# Autodesk Inventor assembly: Ensamblaje SCARA
(part 2 of 2)
- Coincidencia:936 [Mate]: ISO 4017 M4 x 40:3 ↔ ISO 4032 M4:2
- Coincidencia:944 [Mate]: Segundo segmento - inferior - Shape generator prueba 2 - 40%:1 ↔ ISO 7045 H M4 x 16 - 4.8 - H:4
- Coincidencia:945 [Mate]: Segundo segmento - inferior - Shape generator prueba 2 - 40%:1 ↔ ISO 7045 H M4 x 16 - 4.8 - H:5
- Coincidencia:946 [Mate]: Segundo segmento - inferior - Shape generator prueba 2 - 40%:1 ↔ ISO 7045 H M4 x 16 - 4.8 - H:3
- Coincidencia:947 [Mate]: Segundo segmento - inferior - Shape generator prueba 2 - 40%:1 ↔ ISO 7045 H M4 x 16 - 4.8 - H:1
- Coincidencia:948 [Mate]: Segundo segmento - inferior - Shape generator prueba 2 - 40%:1 ↔ ISO 7045 H M4 x 16 - 4.8 - H:2
- Coincidencia:949 [Mate]: Segundo segmento - inferior - Shape generator prueba 2 - 40%:1 ↔ ISO 7045 H M4 x 16 - 4.8 - H:6
- Coincidencia:955 [Mate]: ISO 7045 H M4 x 16 - 4.8 - H:4 ↔ ISO 7089 4:2
- Coincidencia:956 [Mate]: ISO 7045 H M4 x 16 - 4.8 - H:5 ↔ ISO 7089 4:3
- Coincidencia:957 [Mate]: ISO 7045 H M4 x 16 - 4.8 - H:3 ↔ ISO 7089 4:1
- Coincidencia:958 [Mate]: ISO 7045 H M4 x 16 - 4.8 - H:1 ↔ ISO 7089 4:4
- Coincidencia:959 [Mate]: ISO 7045 H M4 x 16 - 4.8 - H:6 ↔ ISO 7089 4:5
- Coincidencia:961 [Mate]: ISO 7045 H M4 x 16 - 4.8 - H:2 ↔ ISO 7089 4:6
- Coincidencia:962 [Mate]: Segundo segmento - inferior - Shape generator prueba 2 - 40%:1 ↔ ISO 7089 4:5
- Coincidencia:963 [Mate]: Segundo segmento - inferior - Shape generator prueba 2 - 40%:1 ↔ ISO 7089 4:6
- Coincidencia:964 [Mate]: Segundo segmento - inferior - Shape generator prueba 2 - 40%:1 ↔ ISO 7089 4:1
- Coincidencia:965 [Mate]: Segundo segmento - inferior - Shape generator prueba 2 - 40%:1 ↔ ISO 7089 4:4
- Coincidencia:966 [Mate]: Segundo segmento - inferior - Shape generator prueba 2 - 40%:1 ↔ ISO 7089 4:3
- Coincidencia:967 [Mate]: Segundo segmento - inferior - Shape generator prueba 2 - 40%:1 ↔ ISO 7089 4:2
- Coincidencia:968 [Mate]: ISO 7045 H M4 x 16 - 4.8 - H:5 ↔ ISO 4032 M4:5
- Coincidencia:969 [Mate]: ISO 7045 H M4 x 16 - 4.8 - H:4 ↔ ISO 4032 M4:6
- Coincidencia:970 [Mate]: ISO 7045 H M4 x 16 - 4.8 - H:3 ↔ ISO 4032 M4:7
- Coincidencia:971 [Mate]: ISO 7045 H M4 x 16 - 4.8 - H:1 ↔ ISO 4032 M4:8
- Coincidencia:972 [Mate]: ISO 7045 H M4 x 16 - 4.8 - H:2 ↔ ISO 4032 M4:9
- Coincidencia:973 [Mate]: ISO 7045 H M4 x 16 - 4.8 - H:6 ↔ ISO 4032 M4:10
- Coincidencia:974 [Mate]: ISO 7089 4:6 ↔ ISO 4032 M4:10
- Coincidencia:975 [Mate]: ISO 4032 M4:7 ↔ ISO 7089 4:4
- Coincidencia:976 [Mate]: ISO 7089 4:6 ↔ ISO 4032 M4:9
- Coincidencia:977 [Mate]: ISO 4032 M4:5 ↔ ISO 7089 4:3
- Coincidencia:978 [Mate]: ISO 4032 M4:6 ↔ ISO 7089 4:2
- Coincidencia:979 [Mate]: ISO 4032 M4:8 ↔ ISO 7089 4:4
- Coincidencia:980 [Mate]: Segundo segmento - inferior - Shape generator prueba 2 - 40%:1 ↔ Segundo segmento - superior:1
- Coincidencia:981 [Mate]: Segundo segmento - inferior - Shape generator prueba 2 - 40%:1 ↔ Segundo segmento - superior:1
- Coincidencia:982 [Mate]: Segundo segmento - inferior - Shape generator prueba 2 - 40%:1 ↔ Segundo segmento - superior:1
- Coincidencia:983 [Mate]: Segundo segmento - superior:1 ↔ Nema+17+Motor+Assembled:6
- Coincidencia:984 [Mate]: Segundo segmento - superior:1 ↔ Nema+17+Motor+Assembled:6
- Coincidencia:985 [Mate]: Segundo segmento - superior:1 ↔ Nema+17+Motor+Assembled:6
- Coincidencia:986 [Mate]: Engranaje para nema 17:5 ↔ Nema+17+Motor+Assembled:6
- Coincidencia:987 [Mate]: Segundo segmento - superior:1 ↔ DIN 625 SKF- con escudo Z SKF 608-Z:10
- Nivelación:115 [Flush]: Segundo segmento - superior:1 ↔ DIN 625 SKF- con escudo Z SKF 608-Z:10
- Coincidencia:988 [Mate]: Segundo segmento - superior:1 ↔ DIN 625 SKF- con escudo Z SKF 608-Z:11
- Nivelación:116 [Flush]: Segundo segmento - superior:1 ↔ DIN 625 SKF- con escudo Z SKF 608-Z:11
- Coincidencia:989 [Mate]: DIN 625 SKF- con escudo Z SKF 608-Z:10 ↔ ISO 2338 8 h8 x 40:4
- Nivelación:117 [Flush]: DIN 625 SKF- con escudo Z SKF 608-Z:10 ↔ ISO 2338 8 h8 x 40:4
- Coincidencia:990 [Mate]: Engrajane doble - primer segmento:3 ↔ ISO 2338 8 h8 x 40:4
- Nivelación:119 [Flush]: Engranaje para nema 17:5 ↔ Engrajane doble - primer segmento:3
- Coincidencia:1000 [Mate]: Segundo segmento - superior:1 ↔ ISO 7045 H M3 x 8 - 4.8 - H:20
- Coincidencia:1001 [Mate]: Segundo segmento - superior:1 ↔ ISO 7045 H M3 x 8 - 4.8 - H:21
- Coincidencia:1002 [Mate]: Segundo segmento - superior:1 ↔ ISO 7045 H M3 x 8 - 4.8 - H:22
- Coincidencia:1003 [Mate]: Segundo segmento - superior:1 ↔ ISO 7045 H M3 x 8 - 4.8 - H:23
- Coincidencia:1004 [Mate]: Segundo segmento - superior:1 ↔ ISO 7045 H M3 x 8 - 4.8 - H:24
- Coincidencia:1005 [Mate]: Segundo segmento - superior:1 ↔ ISO 7045 H M3 x 8 - 4.8 - H:27
- Coincidencia:1006 [Mate]: Segundo segmento - superior:1 ↔ ISO 7045 H M3 x 8 - 4.8 - H:26
- Coincidencia:1007 [Mate]: Segundo segmento - superior:1 ↔ ISO 7045 H M3 x 8 - 4.8 - H:25
- Coincidencia:1008 [Mate]: Segundo segmento - superior:1 ↔ ISO 7045 H M3 x 8 - 4.8 - H:26
- Coincidencia:1009 [Mate]: Segundo segmento - superior:1 ↔ ISO 7045 H M3 x 8 - 4.8 - H:22
- Coincidencia:1010 [Mate]: Segundo segmento - superior:1 ↔ ISO 7045 H M3 x 8 - 4.8 - H:27
- Coincidencia:1011 [Mate]: Segundo segmento - superior:1 ↔ ISO 7045 H M3 x 8 - 4.8 - H:24
- Coincidencia:1012 [Mate]: Segundo segmento - superior:1 ↔ ISO 7045 H M3 x 8 - 4.8 - H:23
- Coincidencia:1013 [Mate]: Segundo segmento - superior:1 ↔ ISO 7045 H M3 x 8 - 4.8 - H:20
- Coincidencia:1014 [Mate]: Segundo segmento - superior:1 ↔ ISO 7045 H M3 x 8 - 4.8 - H:21
- Coincidencia:1015 [Mate]: Segundo segmento - superior:1 ↔ ISO 7045 H M3 x 8 - 4.8 - H:25
- Nivelación:122 [Flush]: Segundo segmento - inferior - Shape generator prueba 2 - 40%:1 ↔ DIN 625 SKF- con escudo Z SKF 608-Z:12
- Coincidencia:1016 [Mate]: Segundo segmento - inferior - Shape generator prueba 2 - 40%:1 ↔ DIN 625 SKF- con escudo Z SKF 608-Z:12
- Coincidencia:1024 [Mate]: ISO 4017 M4 x 40:7 ↔ Engranaje simple - segundo segmento:1
- Coincidencia:1025 [Mate]: ISO 4017 M4 x 40:5 ↔ Engranaje simple - segundo segmento:1
- Coincidencia:1026 [Mate]: ISO 4017 M4 x 40:8 ↔ Engranaje simple - segundo segmento:1
- Coincidencia:1027 [Mate]: ISO 4017 M4 x 40:6 ↔ Engranaje simple - segundo segmento:1
- Nivelación:123 [Flush]: Engrajane doble - primer segmento:3 ↔ Engranaje simple - segundo segmento:1
- Coincidencia:1031 [Mate]: Tercer Segmento - inferior:1 ↔ Tercer segmento - superior:1
- Coincidencia:1032 [Mate]: Tercer Segmento - inferior:1 ↔ Tercer segmento - superior:1
- Coincidencia:1033 [Mate]: Tercer Segmento - inferior:1 ↔ Tercer segmento - superior:1
- Coincidencia:1035 [Mate]: Tercer Segmento - inferior:1 ↔ nema17_pancake:1
- Coincidencia:1036 [Mate]: Tercer Segmento - inferior:1 ↔ nema17_pancake:1
- Coincidencia:1037 [Mate]: Tercer Segmento - inferior:1 ↔ nema17_pancake:1
- Coincidencia:1038 [Mate]: Segundo segmento - inferior - Shape generator prueba 2 - 40%:1 ↔ Joint - Primer segmento:1
- Coincidencia:1039 [Mate]: Primer segmento - superior v1.2:1 ↔ Joint - Primer segmento:1
- Coincidencia:1040 [Mate]: Segundo segmento - inferior - Shape generator prueba 2 - 40%:1 ↔ Joint - Primer segmento:1
- Coincidencia:1041 [Mate]: Primer segmento - superior v1.2:1 ↔ Segundo segmento - inferior - Shape generator prueba 2 - 40%:1
- Coincidencia:1042 [Mate]: Engranaje simple - primer segmento:1 ↔ ISO 4017 M4 x 40:2
- Coincidencia:1043 [Mate]: Engranaje simple - primer segmento:1 ↔ ISO 4017 M4 x 40:1
- Coincidencia:1044 [Mate]: Engranaje simple - primer segmento:1 ↔ ISO 4017 M4 x 40:4
- Coincidencia:1045 [Mate]: Engranaje simple - primer segmento:1 ↔ ISO 4017 M4 x 40:3
- Coincidencia:1046 [Mate]: ISO 4032 M4:1 ↔ Joint - Primer segmento:1
- Coincidencia:1047 [Mate]: ISO 4032 M4:4 ↔ Joint - Primer segmento:1
- Coincidencia:1048 [Mate]: ISO 4032 M4:2 ↔ Joint - Primer segmento:1
- Coincidencia:1049 [Mate]: ISO 4032 M4:3 ↔ Joint - Primer segmento:1
- Coincidencia:1050 [Mate]: ISO 7045 H M4 x 16 - 4.8 - H:6 ↔ Joint - Primer segmento:1
- Coincidencia:1051 [Mate]: ISO 7045 H M4 x 16 - 4.8 - H:3 ↔ Joint - Primer segmento:1
- Coincidencia:1052 [Mate]: ISO 7045 H M4 x 16 - 4.8 - H:2 ↔ Joint - Primer segmento:1
- Coincidencia:1053 [Mate]: ISO 7045 H M4 x 16 - 4.8 - H:1 ↔ Joint - Primer segmento:1
- Coincidencia:1054 [Mate]: ISO 7045 H M4 x 16 - 4.8 - H:4 ↔ Joint - Primer segmento:1
- Coincidencia:1055 [Mate]: ISO 7045 H M4 x 16 - 4.8 - H:5 ↔ Joint - Primer segmento:1
- Coincidencia:1056 [Mate]: ISO 7045 H M4 x 16 - 4.8 - H:6 ↔ Joint - Primer segmento:1
- Coincidencia:1057 [Mate]: ISO 7045 H M4 x 16 - 4.8 - H:1 ↔ Joint - Primer segmento:1
- Coincidencia:1058 [Mate]: ISO 7045 H M4 x 16 - 4.8 - H:3 ↔ Joint - Primer segmento:1
- Coincidencia:1059 [Mate]: ISO 7045 H M4 x 16 - 4.8 - H:4 ↔ Joint - Primer segmento:1
- Coincidencia:1060 [Mate]: ISO 7045 H M4 x 16 - 4.8 - H:5 ↔ Joint - Primer segmento:1
- Coincidencia:1061 [Mate]: ISO 7045 H M4 x 16 - 4.8 - H:2 ↔ Joint - Primer segmento:1
- Coincidencia:1062 [Mate]: Segundo segmento - superior:1 ↔ JIS B 1521 6805 25x37x7:5
- Coincidencia:1063 [Mate]: Segundo segmento - inferior - Shape generator prueba 2 - 40%:1 ↔ JIS B 1521 6805 25x37x7:5
- Coincidencia:1064 [Mate]: Engranaje simple - segundo segmento:1 ↔ JIS B 1521 6805 25x37x7:5
- Coincidencia:1065 [Mate]: JIS B 1521 6805 25x37x7:5 ↔ Joint - Segundo segmento:1
- Coincidencia:1066 [Mate]: Engranaje simple - segundo segmento:1 ↔ Joint - Segundo segmento:1
- Coincidencia:1067 [Mate]: Engranaje simple - segundo segmento:1 ↔ Joint - Segundo segmento:1
- Coincidencia:1068 [Mate]: Tercer segmento - superior:1 ↔ Joint - Segundo segmento:1
- Coincidencia:1069 [Mate]: Tercer segmento - superior:1 ↔ Joint - Segundo segmento:1
- Coincidencia:1070 [Mate]: Tercer segmento - superior:1 ↔ Joint - Segundo segmento:1
- Coincidencia:1071 [Mate]: ISO 4017 M4 x 40:5 ↔ ISO 4032 M4:14
- Coincidencia:1072 [Mate]: ISO 4017 M4 x 40:8 ↔ ISO 4032 M4:13
- Coincidencia:1073 [Mate]: ISO 4017 M4 x 40:6 ↔ ISO 4032 M4:11
- Coincidencia:1074 [Mate]: ISO 4017 M4 x 40:7 ↔ ISO 4032 M4:12
- Coincidencia:1075 [Mate]: ISO 4017 M4 x 40:8 ↔ Joint - Segundo segmento:1
- Coincidencia:1076 [Mate]: ISO 4017 M4 x 40:6 ↔ Joint - Segundo segmento:1
- Coincidencia:1077 [Mate]: ISO 4017 M4 x 40:7 ↔ Joint - Segundo segmento:1
- Coincidencia:1078 [Mate]: ISO 4017 M4 x 40:5 ↔ Joint - Segundo segmento:1
- Coincidencia:1079 [Mate]: Joint - Segundo segmento:1 ↔ ISO 4032 M4:13
- Coincidencia:1080 [Mate]: Joint - Segundo segmento:1 ↔ ISO 4032 M4:14
- Coincidencia:1081 [Mate]: Joint - Segundo segmento:1 ↔ ISO 4032 M4:11
- Coincidencia:1082 [Mate]: Joint - Segundo segmento:1 ↔ ISO 4032 M4:12
- [Mate]: ISO 7045 H M4 x 16 - 4.8 - H:7 ↔ ISO 7089 4:7
- [Mate]: ISO 7045 H M4 x 16 - 4.8 - H:7 ↔ ISO 4032 M4:15
- [Mate]: ISO 7045 H M4 x 16 - 4.8 - H:8 ↔ ISO 7089 4:8
- [Mate]: ISO 7045 H M4 x 16 - 4.8 - H:8 ↔ ISO 4032 M4:16
- [Mate]: ISO 7045 H M4 x 16 - 4.8 - H:10 ↔ ISO 7089 4:10
- [Mate]: ISO 7045 H M4 x 16 - 4.8 - H:10 ↔ ISO 4032 M4:18
- [Mate]: ISO 7045 H M4 x 16 - 4.8 - H:11 ↔ ISO 7089 4:11
- [Mate]: ISO 7045 H M4 x 16 - 4.8 - H:11 ↔ ISO 4032 M4:19
- [Mate]: ISO 7045 H M4 x 16 - 4.8 - H:12 ↔ ISO 7089 4:12
- [Mate]: ISO 7045 H M4 x 16 - 4.8 - H:12 ↔ ISO 4032 M4:20
- Coincidencia:1095 [Mate]: Joint - Segundo segmento:1 ↔ ISO 7045 H M4 x 16 - 4.8 - H:12
- Coincidencia:1096 [Mate]: Joint - Segundo segmento:1 ↔ ISO 7045 H M4 x 16 - 4.8 - H:11
- Coincidencia:1097 [Mate]: Joint - Segundo segmento:1 ↔ ISO 7045 H M4 x 16 - 4.8 - H:8
- Coincidencia:1098 [Mate]: Joint - Segundo segmento:1 ↔ ISO 7045 H M4 x 16 - 4.8 - H:7
- [Mate]: ISO 7045 H M4 x 16 - 4.8 - H:14 ↔ ISO 7089 4:14
- [Mate]: ISO 7045 H M4 x 16 - 4.8 - H:14 ↔ ISO 4032 M4:22
- Coincidencia:1103 [Mate]: Joint - Segundo segmento:1 ↔ ISO 7045 H M4 x 16 - 4.8 - H:14
- Coincidencia:1104 [Mate]: Joint - Segundo segmento:1 ↔ ISO 7045 H M4 x 16 - 4.8 - H:10
- Coincidencia:1105 [Mate]: Joint - Segundo segmento:1 ↔ ISO 7045 H M4 x 16 - 4.8 - H:7
- Coincidencia:1106 [Mate]: Joint - Segundo segmento:1 ↔ ISO 7045 H M4 x 16 - 4.8 - H:8
- Coincidencia:1107 [Mate]: Joint - Segundo segmento:1 ↔ ISO 7045 H M4 x 16 - 4.8 - H:12
- Coincidencia:1108 [Mate]: Joint - Segundo segmento:1 ↔ ISO 7045 H M4 x 16 - 4.8 - H:11
- Coincidencia:1109 [Mate]: Joint - Segundo segmento:1 ↔ ISO 7045 H M4 x 16 - 4.8 - H:14
- Coincidencia:1110 [Mate]: Joint - Segundo segmento:1 ↔ ISO 7045 H M4 x 16 - 4.8 - H:10
- Coincidencia:1111 [Mate]: Tercer segmento - superior:1 ↔ ISO 7089 4:10
- Coincidencia:1112 [Mate]: ISO 7089 4:10 ↔ ISO 4032 M4:18
- Coincidencia:1113 [Mate]: Tercer segmento - superior:1 ↔ ISO 7089 4:14
- Coincidencia:1114 [Mate]: Tercer segmento - superior:1 ↔ ISO 7089 4:7
- Coincidencia:1115 [Mate]: Tercer segmento - superior:1 ↔ ISO 7089 4:8
- Coincidencia:1116 [Mate]: Tercer segmento - superior:1 ↔ ISO 7089 4:11
- Coincidencia:1117 [Mate]: Tercer segmento - superior:1 ↔ ISO 7089 4:12
- Coincidencia:1118 [Mate]: ISO 7089 4:11 ↔ ISO 4032 M4:20
- Coincidencia:1119 [Mate]: ISO 7089 4:8 ↔ ISO 4032 M4:16
- Coincidencia:1120 [Mate]: ISO 7089 4:7 ↔ ISO 4032 M4:15
- Coincidencia:1121 [Mate]: ISO 7089 4:14 ↔ ISO 4032 M4:22
- Coincidencia:1122 [Mate]: ISO 7089 4:11 ↔ ISO 4032 M4:19
- Coincidencia:1126 [Mate]: nema17_pancake:1 ↔ Engranaje para nema 17:6
- Coincidencia:1127 [Mate]: Tercer Segmento - inferior:1 ↔ Tercer segmento - superior:1
- [Mate]: ISO 4014 M3 x 20:3 ↔ Polea Lisa - eje3mm:3
- [Mate]: ISO 4014 M3 x 20:3 ↔ ISO 7089 3:9
- [Mate]: ISO 4014 M3 x 20:3 ↔ ISO 4032 M3:11
- [Mate]: ISO 4014 M3 x 20:3 ↔ ISO 4032 M3:12
- [Mate]: ISO 4014 M3 x 20:3 ↔ Polea Lisa - eje3mm:3
- [Mate]: ISO 4032 M3:11 ↔ ISO 7089 3:9
- [Mate]: Polea Lisa - eje3mm:3 ↔ ISO 4032 M3:11
- Coincidencia:1143 [Mate]: Segundo segmento - inferior - Shape generator prueba 2 - 40%:1 ↔ ISO 7089 3:9
- Coincidencia:1144 [Mate]: Segundo segmento - inferior - Shape generator prueba 2 - 40%:1 ↔ ISO 4032 M3:12
- Coincidencia:1145 [Mate]: Segundo segmento - inferior - Shape generator prueba 2 - 40%:1 ↔ ISO 7089 3:9
- [Mate]: ISO 4014 M3 x 20:4 ↔ Polea Lisa - eje3mm:4
- [Mate]: ISO 4014 M3 x 20:4 ↔ ISO 7089 3:10
- [Mate]: ISO 4014 M3 x 20:4 ↔ ISO 4032 M3:13
- [Mate]: ISO 4014 M3 x 20:4 ↔ ISO 4032 M3:14
- [Mate]: ISO 4014 M3 x 20:4 ↔ Polea Lisa - eje3mm:4
- [Mate]: ISO 4032 M3:13 ↔ ISO 7089 3:10
- [Mate]: Polea Lisa - eje3mm:4 ↔ ISO 4032 M3:13
- [Mate]: ISO 4014 M3 x 20:5 ↔ Polea Lisa - eje3mm:5
- [Mate]: ISO 4014 M3 x 20:5 ↔ ISO 7089 3:11
- [Mate]: ISO 4014 M3 x 20:5 ↔ ISO 4032 M3:15
- [Mate]: ISO 4014 M3 x 20:5 ↔ ISO 4032 M3:16
- [Mate]: ISO 4014 M3 x 20:5 ↔ Polea Lisa - eje3mm:5
- [Mate]: ISO 4032 M3:15 ↔ ISO 7089 3:11
- [Mate]: Polea Lisa - eje3mm:5 ↔ ISO 4032 M3:15
- Nivelación:126 [Flush]: Polea Lisa - eje3mm:4 ↔ Polea Lisa - eje3mm:5
- Coincidencia:1160 [Mate]: Tercer Segmento - inferior:1 ↔ ISO 4014 M3 x 20:4
- Coincidencia:1161 [Mate]: Tercer Segmento - inferior:1 ↔ ISO 4014 M3 x 20:5
- Coincidencia:1162 [Mate]: Tercer Segmento - inferior:1 ↔ JIS B 1521 6805 25x37x7:6
- Nivelación:127 [Flush]: Tercer Segmento - inferior:1 ↔ JIS B 1521 6805 25x37x7:6
- Coincidencia:1163 [Mate]: Engranaje simple - segundo segmento:2 ↔ JIS B 1521 6805 25x37x7:6
- Coincidencia:1164 [Mate]: Engranaje simple - segundo segmento:2 ↔ JIS B 1521 6805 25x37x7:6
- Coincidencia:1165 [Mate]: Tercer Segmento - inferior:1 ↔ ISO 7089 3:10
- Coincidencia:1166 [Mate]: Tercer Segmento - inferior:1 ↔ ISO 4032 M3:16
- Ángulo:30 [Angle] (0 deg): Tercer Segmento - inferior:1 ↔ ISO 4032 M3:16
- Coincidencia:1167 [Mate]: Tercer Segmento - inferior:1 ↔ ISO 4032 M3:14
- Nivelación:128 [Flush]: Engranaje para nema 17:6 ↔ Engranaje simple - segundo segmento:2
- Coincidencia:1168 [Mate]: Tercer Segmento - inferior:1 ↔ ISO 7045 H M3 x 8 - 4.8 - H:28
- Coincidencia:1169 [Mate]: Tercer Segmento - inferior:1 ↔ ISO 7045 H M3 x 8 - 4.8 - H:29
- Coincidencia:1170 [Mate]: Tercer Segmento - inferior:1 ↔ ISO 7045 H M3 x 8 - 4.8 - H:30
- Coincidencia:1171 [Mate]: Tercer Segmento - inferior:1 ↔ ISO 7045 H M3 x 8 - 4.8 - H:31
- Coincidencia:1172 [Mate]: Tercer Segmento - inferior:1 ↔ ISO 7045 H M3 x 8 - 4.8 - H:35
- Coincidencia:1173 [Mate]: Tercer Segmento - inferior:1 ↔ ISO 7045 H M3 x 8 - 4.8 - H:34
- Coincidencia:1174 [Mate]: Tercer Segmento - inferior:1 ↔ ISO 7045 H M3 x 8 - 4.8 - H:32
- Coincidencia:1175 [Mate]: Tercer Segmento - inferior:1 ↔ ISO 7045 H M3 x 8 - 4.8 - H:33
- Coincidencia:1176 [Mate]: Tercer Segmento - inferior:1 ↔ ISO 7045 H M3 x 8 - 4.8 - H:31
- Coincidencia:1177 [Mate]: Tercer Segmento - inferior:1 ↔ ISO 7045 H M3 x 8 - 4.8 - H:35
- Coincidencia:1178 [Mate]: Tercer Segmento - inferior:1 ↔ ISO 7045 H M3 x 8 - 4.8 - H:30
- Coincidencia:1179 [Mate]: Tercer Segmento - inferior:1 ↔ ISO 7045 H M3 x 8 - 4.8 - H:34
- Coincidencia:1180 [Mate]: Tercer Segmento - inferior:1 ↔ ISO 7045 H M3 x 8 - 4.8 - H:29
- Coincidencia:1181 [Mate]: Tercer Segmento - inferior:1 ↔ ISO 7045 H M3 x 8 - 4.8 - H:32
- Coincidencia:1182 [Mate]: Tercer Segmento - inferior:1 ↔ ISO 7045 H M3 x 8 - 4.8 - H:28
- Coincidencia:1183 [Mate]: Tercer Segmento - inferior:1 ↔ ISO 7045 H M3 x 8 - 4.8 - H:33
- Coincidencia:1184 [Mate]: ISO 4017 M4 x 40:3 ↔ Joint - Primer segmento:1
- Coincidencia:1191 [Mate]: Tercer segmento - superior:1 ↔ DIN 625 SKF- con escudo Z SKF 608-Z:13
- Nivelación:131 [Flush]: Tercer segmento - superior:1 ↔ DIN 625 SKF- con escudo Z SKF 608-Z:13
- Coincidencia:1197 [Mate]: DIN 625 SKF- con escudo Z SKF 608-Z:9 ↔ ISO 2338 8 h8 x 50:1
- Nivelación:133 [Flush]: DIN 625 SKF- con escudo Z SKF 608-Z:9 ↔ ISO 2338 8 h8 x 50:1
- Coincidencia:1198 [Mate]: DIN 625 SKF- con escudo Z SKF 608-Z:11 ↔ ISO 2338 8 h8 x 50:2
- Nivelación:134 [Flush]: DIN 625 SKF- con escudo Z SKF 608-Z:11 ↔ ISO 2338 8 h8 x 50:2
- Coincidencia:1199 [Mate]: DIN 625 SKF- con escudo Z SKF 608-Z:13 ↔ ISO 2338 8 h8 x 30:1
- Nivelación:135 [Flush]: DIN 625 SKF- con escudo Z SKF 608-Z:13 ↔ ISO 2338 8 h8 x 30:1
- Coincidencia:1207 [Mate]: Base - Gripper:1 ↔ Servo SG90:1
- Coincidencia:1208 [Mate]: Base - Gripper:1 ↔ Servo SG90:1
- Coincidencia:1209 [Mate]: Base - Gripper:1 ↔ Servo SG90:1
- Coincidencia:1210 [Mate]: roue dentée 38B1:1 ↔ Base - Gripper:1
- Coincidencia:1211 [Mate]: Base - Gripper:1 ↔ Logitech c270:1
- Coincidencia:1212 [Mate]: Base - Gripper:1 ↔ Logitech c270:1
- Coincidencia:1213 [Mate]: roue dentée 38A1:1 ↔ Servo SG90:1
- Nivelación:136 [Flush]: roue dentée 38A1:1 ↔ Servo SG90:1
- Coincidencia:1214 [Mate]: Base - version 2:1 ↔ Servo SG90:2
- Ángulo:31 [Angle] (0 deg): Base - version 2:1 ↔ Servo SG90:2
- Coincidencia:1215 [Mate]: Base - version 2:1 ↔ Servo SG90:2
- Coincidencia:1216 [Mate]: Round_gear:1 ↔ Servo SG90:2
- Nivelación:137 [Flush] (-5.6 mm): Round_gear:1 ↔ Servo SG90:2
- Coincidencia:1217 [Mate]: Base - version 2:1 ↔ Logitech c270:2
- Ángulo:32 [Angle] (180 deg): Base - version 2:1 ↔ Logitech c270:2
- Coincidencia:1218 [Mate]: Base - version 2:1 ↔ Logitech c270:2
- Coincidencia:1219 [Mate]: Base - version 2:1 ↔ Tapa - Gripper:1
- Coincidencia:1220 [Mate]: Base - version 2:1 ↔ Tapa - Gripper:1
- Coincidencia:1221 [Mate]: Base - version 2:1 ↔ Tapa - Gripper:1
- Coincidencia:1222 [Mate]: Engranaje simple - segundo segmento:2 ↔ Tapa - Gripper:1
- Coincidencia:1223 [Mate]: Engranaje simple - segundo segmento:2 ↔ Tapa - Gripper:1
- Coincidencia:1228 [Mate]: Base - version 2:1 ↔ Pata derecha - versión 3:1
- Coincidencia:1229 [Mate]: Base - version 2:1 ↔ Pata derecha - versión 3:1
- Coincidencia:1230 [Mate]: Base - version 2:1 ↔ Pata Izquierda - versión 3:1
- Coincidencia:1231 [Mate]: Base - version 2:1 ↔ Pata Izquierda - versión 3:1
- Coincidencia:1232 [Mate]: Pata Izquierda - versión 3:1 ↔ Base Marcador ECU + Gripper:1
- Ángulo:33 [Angle] (0 deg): Pata Izquierda - versión 3:1 ↔ Base Marcador ECU + Gripper:1
- Coincidencia:1233 [Mate]: Segundo segmento - inferior - Shape generator prueba 2 - 40%:1 ↔ ISO 4014 M3 x 20:3
- Coincidencia:1234 [Mate]: Segundo segmento - inferior - Shape generator prueba 2 - 40%:1 ↔ ISO 7089 3:9
- Coincidencia:1235 [Mate] (3 mm): Perfil 2040 200 mm v4:3 ↔ Soporte del primer segmento:2
- Nivelación:138 [Flush] (-20 mm): Perfil 2040 200 mm v4:3 ↔ Soporte del primer segmento:2
- Coincidencia:1236 [Mate]: Engranaje simple - segundo segmento:2 ↔ Tapa - Gripper:1
- Coincidencia:1237 [Mate]: Tercer Segmento - inferior:1 ↔ ISO 7089 3:10
## Named parameters: d145_d66_d56_d24_d16 = 0 mm, d146_d67_d57_d25_d17 = 0 mm, d147_d68_d58_d26_d18 = 0 mm, d148_d69_d59_d27_d19 = 0 mm, d776_d729 = 0 mm, d777_d730 = 0 mm, d778_d731 = 0 mm, d779_d737 = 0 mm, d780_d739 = 0 mm, d781_d740 = 0 mm, d782_d741 = 0 mm, d783_d742 = 0 mm, d784_d743 = 0 mm, d785_d744 = 0 mm, d786_d745 = 0 mm, d787_d746 = 0 mm, d788_d747 = 0 mm, d789_d748 = 0 mm, d790_d749 = 0 mm, d791_d750 = 0 mm, d792_d751 = 0 mm, d1304_d1107 = 0 mm, d1305_d1108 = 0 mm, d1306_d1109 = 0 mm, d1307_d1110 = 0 mm, d1308_d1111 = 0 mm, d1309_d1112 = 0 mm, d1310_d1113 = 0 mm, d1311_d1114 = 0 mm, d1312_d1115 = 0 mm, d1313_d1116 = 0 mm, d1314_d1117 = 0 mm, d1315_d1118 = 0 mm, d1316_d1119 = 0 mm, d1317_d1124 = 0 mm, d1318_d1125 = 0 mm, d1319_d1126 = 0 mm, d1320_d1177 = 0 mm, d1321_d1105 = 0 mm, d1322_d1106 = 0 mm, d1323_d1003 = 0 mm, d1324_d1004 = 0 deg, d1325_d1006 = 0 mm, d1326_d1007 = 0 mm, d1327_d1008 = 0 deg, d1328_d960_d461_d287_d239_d204 = 0 mm, d1329_d961_d462_d288_d240_d205 = 0 mm, d1330_d962_d463_d290_d242_d66_d56_d24_d16 = 0 mm, d1331_d963_d464_d291_d243_d67_d57_d25_d17 = 0 mm, d1332_d964_d465_d292_d244_d68_d58_d26_d18 = 0 mm, d1333_d965_d466_d293_d245_d69_d59_d27_d19 = 0 mm, d1334_d966_d467_d294_d246_d216 = 0 mm, d1335_d967_d468_d296_d248_d218 = 0 mm, d1336_d968_d470_d298_d250 = 0 mm, d1337_d969_d471_d458 = 0 mm, d1338_d970_d472_d459 = 0 mm, d1339_d971_d461_d287_d239_d204 = 0 mm, d1340_d972_d462_d288_d240_d205 = 0 mm, d1341_d973_d463_d290_d242_d66_d56_d24_d16 = 0 mm, d1342_d974_d464_d291_d243_d67_d57_d25_d17 = 0 mm, d1343_d975_d465_d292_d244_d68_d58_d26_d18 = 0 mm, d1344_d976_d466_d293_d245_d69_d59_d27_d19 = 0 mm, d1345_d977_d467_d294_d246_d216 = 0 mm, d1346_d978_d468_d296_d248_d218 = 0 mm, d1347_d979_d470_d298_d250 = 0 mm, d1348_d980_d471_d458 = 0 mm, d1349_d981_d472_d459 = 0 mm, d1350_d982_d461_d287_d239_d204 = 0 mm, d1351_d983_d462_d288_d240_d205 = 0 mm, d1352_d984_d463_d290_d242_d66_d56_d24_d16 = 0 mm, d1353_d985_d464_d291_d243_d67_d57_d25_d17 = 0 mm, d1354_d986_d465_d292_d244_d68_d58_d26_d18 = 0 mm, d1355_d987_d466_d293_d245_d69_d59_d27_d19 = 0 mm, d1356_d988_d467_d294_d246_d216 = 0 mm, d1357_d989_d468_d296_d248_d218 = 0 mm, d1358_d990_d470_d298_d250 = 0 mm, d1359_d991_d471_d458 = 0 mm, d1360_d992_d472_d459 = 0 mm, d1361_d993 = 0 mm, d1362_d994 = 0 mm, d1363_d995 = 0 deg, d1364_d996 = 0 mm, d1365_d997 = 0 mm, d1366_d998 = 0 mm, d1367_d999 = 0 mm, d1368_d1000 = 0 deg, d1369_d1002 = 0 mm, d1370_d949_d461_d287_d239_d204 = 0 mm, d1371_d950_d462_d288_d240_d205 = 0 mm, d1372_d951_d463_d290_d242_d66_d56_d24_d16 = 0 mm, d1373_d952_d464_d291_d243_d67_d57_d25_d17 = 0 mm, d1374_d953_d465_d292_d244_d68_d58_d26_d18 = 0 mm, d1375_d954_d466_d293_d245_d69_d59_d27_d19 = 0 mm, d1376_d955_d467_d294_d246_d216 = 0 mm, d1377_d956_d468_d296_d248_d218 = 0 mm, d1378_d957_d470_d298_d250 = 0 mm, d1379_d958_d471_d458 = 0 mm, d1380_d959_d472_d459 = 0 mm, d1381_d525 = 0 mm, d1382_d526 = 0 mm, d1383_d527 = 0 mm, d1384_d528 = 0 mm, d1385_d529 = 0 mm, d1386_d530 = 0 mm, d1387_d447 = 0 mm, d1388_d448 = 0 mm, d1389_d449 = 0 mm, d1390_d450 = 0 mm, d1391_d452 = 0 mm, d1392_d453 = 0 mm, d1393_d454 = 0 mm, d1394_d455 = 0 mm, d1395_d456 = 0 mm, d1396_d457 = 0 mm, d1397_d460_d344 = 0 mm, d1398_d461_d287_d239_d204 = 0 mm, d1399_d462_d288_d240_d205 = 0 mm, d1400_d463_d290_d242_d66_d56_d24_d16 = 0 mm, d1401_d464_d291_d243_d67_d57_d25_d17 = 0 mm, d1402_d465_d292_d244_d68_d58_d26_d18 = 0 mm, d1403_d466_d293_d245_d69_d59_d27_d19 = 0 mm, d1404_d467_d294_d246_d216 = 0 mm, d1405_d468_d296_d248_d218 = 0 mm, d1406_d469_d297_d249 = 0 mm, d1407_d470_d298_d250 = 0 mm, d1408_d471_d458 = 0 mm, d1409_d472_d459 = 0 mm, d1410_d512_d344 = 0 mm, d1411_d513_d287_d239_d204 = 0 mm, d1412_d514_d288_d240_d205 = 0 mm, d1413_d515_d290_d242_d66_d56_d24_d16 = 0 mm, d1414_d516_d291_d243_d67_d57_d25_d17 = 0 mm, d1415_d517_d292_d244_d68_d58_d26_d18 = 0 mm, d1416_d518_d293_d245_d69_d59_d27_d19 = 0 mm, d1417_d519_d294_d246_d216 = 0 mm, d1418_d520_d296_d248_d218 = 0 mm, d1419_d521_d297_d249 = 0 mm, d1420_d522_d298_d250 = 0 mm, d1421_d523_d458 = 0 mm, d1422_d524_d459 = 0 mm, d1423_d218 = 0 mm, d1424_d311_d239_d204 = 0 mm, d1425_d312_d240_d205 = 0 mm, d1426_d314_d242_d66_d56_d24_d16 = 0 mm, d1427_d315_d243_d67_d57_d25_d17 = 0 mm, d1428_d316_d244_d68_d58_d26_d18 = 0 mm, d1429_d317_d245_d69_d59_d27_d19 = 0 mm, d1430_d318_d246_d216 = 0 mm, d1431_d320_d248_d218 = 0 mm, d1432_d321_d249 = 0 mm, d1433_d322_d250 = 0 mm, d1434_d323 = 0 mm, d1435_d325 = 0 mm, d1436_d326 = 0 mm, d1437_d330 = 0 mm, d1438_d66_d56_d24_d16 = 0 mm, d1439_d67_d57_d25_d17 = 0 mm, d1440_d68_d58_d26_d18 = 0 mm, d1441_d69_d59_d27_d19 = 0 mm, d1442_d204 = 0 mm, d1443_d205 = 0 mm, d1444_d216 = 0 mm, d1687_d1545 = 0 mm, d1688_d1559 = 0 mm, d1689_d1545 = 0 mm, d1690_d1559 = 0 mm, d1693_d1545 = 0 mm, d1694_d1559 = 0 mm, d1695_d1545 = 0 mm, d1696_d1559 = 0 mm, d1697_d1545 = 0 mm, d1698_d1559 = 0 mm, d1705_d1545 = 0 mm, d1706_d1559 = 0 mm, d1742_d1734_d1034 = 0 mm, d1743_d1735_d1035 = 0 mm, d1744_d1736_d1036 = 0 mm, d1745_d1737_d1037 = 0 mm, d1746_d1738_d1038 = 0 mm, d1747_d1739_d1039 = 0 mm, d1748_d1740_d1040 = 0 mm, d1759_d1734_d1034 = 0 mm, d1760_d1735_d1035 = 0 mm, d1761_d1736_d1036 = 0 mm, d1762_d1737_d1037 = 0 mm, d1763_d1738_d1038 = 0 mm, d1764_d1739_d1039 = 0 mm, d1765_d1740_d1040 = 0 mm, d1766_d1734_d1034 = 0 mm, d1767_d1735_d1035 = 0 mm, d1768_d1736_d1036 = 0 mm, d1769_d1737_d1037 = 0 mm, d1770_d1738_d1038 = 0 mm, d1771_d1739_d1039 = 0 mm, d1772_d1740_d1040 = 0 mm
